# Autodesk Inventor assembly: Orbital motor with mounts
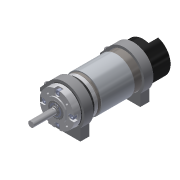
[picture p0: Inventor's stored thumbnail of the model, 180x180]
Saved by Autodesk Inventor 2018 (Build 220112000, 112)
## iProperties
Created: 2019-01-13
Part Number: Orbital motor with mounts
Document SubType Name: Assembly
Designer: ball
Author: ball
## Documents named in this file (3)
- C:\FTC\FTC8863CAD\Andymark\Orbital motor with mounts.iam
- C:\FTC\FTC8863CAD\Andymark\am-3461a NeveRest 4 with Motor REV3.ipt
- C:\FTC\FTC8863CAD\Actobotics\555 parts\555116 assembly.ipt
## Components (3 placed, 2 different names)
1. am-3461a NeveRest 4 with Motor REV3:1 — Mate:1, Mate:2, Flush:1, Flush:2
2. 555116 assembly:1 — Mate:1, Flush:1, Flush:3
3. 555116 assembly:2 — Mate:2, Flush:2, Flush:3
## Relationships (5: Flush 3, Mate 2)
- Mate:1: am-3461a NeveRest 4 with Motor REV3:1 ↔ 555116 assembly:1
- Mate:2: am-3461a NeveRest 4 with Motor REV3:1 ↔ 555116 assembly:2
- Flush:1 (7.62 mm): am-3461a NeveRest 4 with Motor REV3:1 ↔ 555116 assembly:1
- Flush:2 (-20.32 mm): am-3461a NeveRest 4 with Motor REV3:1 ↔ 555116 assembly:2
- Flush:3: 555116 assembly:1 ↔ 555116 assembly:2
